# Autodesk Inventor assembly: Kitv2
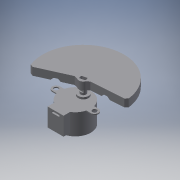
[picture p0: Inventor's stored thumbnail of the model, 180x180]
Saved by Autodesk Inventor 2018.3 (Build 223284000, 284)
## iProperties
Created: 2019-02-23
Part Number: Kitv2
Material: 一般
Document SubType Name: Assembly
Designer: shun2
Author: shun2
## Documents named in this file (3)
- C:\Users\shun2\OneDrive\おそらく最新版(2018.7.31)\レスキューキット投下機構\Kitv2.iam
- C:\Users\shun2\OneDrive\おそらく最新版(2018.7.31)\レスキューキット投下機構\28BYJ-48.ipt
- C:\Users\shun2\OneDrive\おそらく最新版(2018.7.31)\レスキューキット投下機構\RescueKitThrow-Joint.ipt
## Components (2 placed, 2 different names)
1. 28BYJ-48:1 — メイト:1, フラッシュ:1
2. RescueKitThrow-Joint:1 — メイト:1, フラッシュ:1
## Relationships (2: Mate 1, Flush 1)
- メイト:1 [Mate]: 28BYJ-48:1 ↔ RescueKitThrow-Joint:1
- フラッシュ:1 [Flush] (-3.759 mm): 28BYJ-48:1 ↔ RescueKitThrow-Joint:1
